# Autodesk Inventor assembly: batteryHolderAssembly
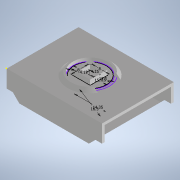
[picture p0: Inventor's stored thumbnail of the model, 180x180]
Saved by Autodesk Inventor 2022 (Build 260153000, 153)
## iProperties
Created: 2022-08-09
Part Number: batteryHolderAssembly
Document SubType Name: Assembly
Designer: sgioj
Mass: 4.89416 g
Surface Area: 84.1239 cm^2
Volume: 4.89416 cm^3
Density: 1 g/cm^3
Author: sgioj
## Documents named in this file (4)
- C:\Autodesk\wirelessLights\batteryHolderAssembly.iam
- C:\Autodesk\wirelessLights\ButtonBatteryHolder.ipt
- C:\Autodesk\wirelessLights\buttonBatteryConnector.ipt
- C:\Autodesk\wirelessLights\pwrButton.ipt
## Components (3 placed, 3 different names)
1. ButtonBatteryHolder:1 — Insert:1, Insert:2
2. buttonBatteryConnector:1 — Insert:1
3. pwrButton:1 — Insert:2
## Relationships (2: Insert 2)
- Insert:1: ButtonBatteryHolder:1 ↔ buttonBatteryConnector:1
- Insert:2: ButtonBatteryHolder:1 ↔ pwrButton:1
